# Autodesk Inventor assembly: SE Base Matriz Centelladora DC
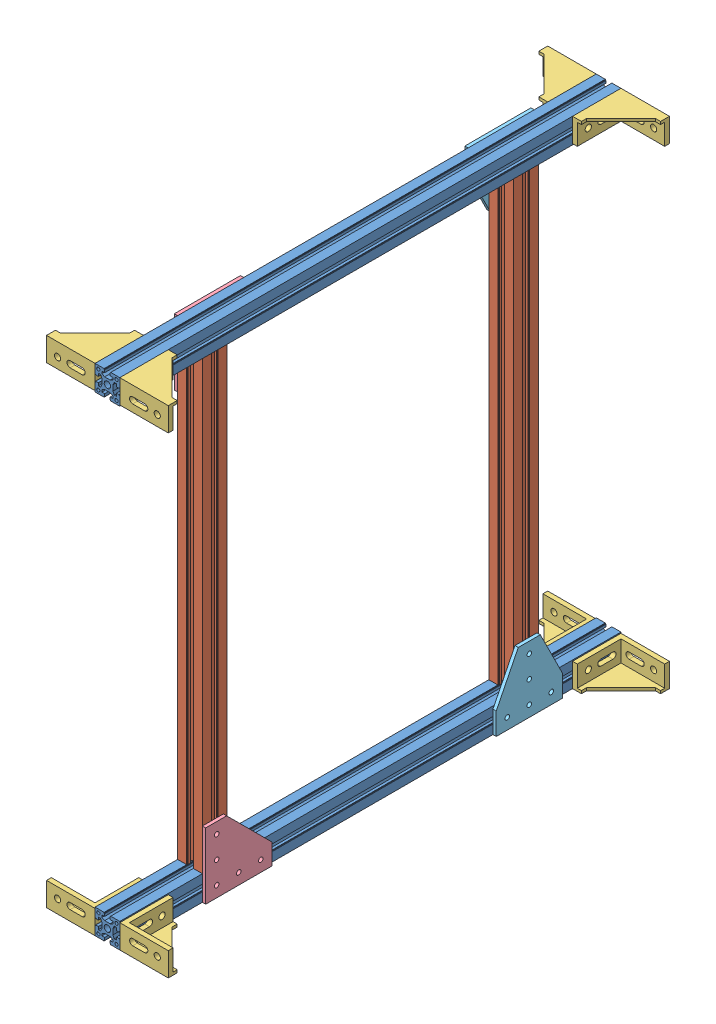
[picture p0: shaded view drawn from the part files that the assembly names]
Saved by Autodesk Inventor 2024.2 (Build 282272000, 272)
## iProperties
Created: 2025-11-13
Part Number: SE Base Matriz Centelladora DC
Document SubType Name: Assembly
Designer: ja.restrepo1
Author: ja.restrepo1
## Documents named in this file (7)
- I:\MICROMECANICA\ALTAS ENERGIAS\Deteccion de Muones\Detectores centelladores\Partes Detector Centellador\SE Base Matriz Centelladora DC\SE Base Matriz Centelladora DC.iam
- I:\MICROMECANICA\ALTAS ENERGIAS\Deteccion de Muones\Detectores centelladores\Partes Detector Centellador\SE Chasis DC\Partes Chasis DC\Perfil 45X45\Perfil 45X45x910.ipt
- I:\MICROMECANICA\ALTAS ENERGIAS\Deteccion de Muones\Detectores centelladores\Partes Detector Centellador\SE Chasis DC\Partes Chasis DC\Perfil 45X45.ipt
- I:\MICROMECANICA\ALTAS ENERGIAS\Deteccion de Muones\Detectores centelladores\Partes Detector Centellador\SE Chasis DC\Partes Chasis DC\Perfil 45X45\Perfil 45X45X810.ipt
- I:\MICROMECANICA\ALTAS ENERGIAS\Deteccion de Muones\Detectores centelladores\Partes Detector Centellador\SE Chasis DC\Partes Chasis DC\Accesorios perfileria\escuadra grande.ipt
- I:\MICROMECANICA\ALTAS ENERGIAS\Deteccion de Muones\Detectores centelladores\Partes Detector Centellador\SE Chasis DC\Partes Chasis DC\Accesorios perfileria\escuadra plana.ipt
- I:\MICROMECANICA\ALTAS ENERGIAS\Deteccion de Muones\Detectores centelladores\Partes Detector Centellador\SE Chasis DC\Partes Chasis DC\Accesorios perfileria\T.ipt
## Components (16 placed, 5 different names)
1. Perfil 45X45x910:1 — Flush:19, Flush:20, Flush:21, Flush:22, Flush:23, Flush:24, Flush:25, Flush:26
2. Perfil 45X45x910:2 — Flush:19, Flush:27, Flush:28, Flush:29, Flush:30
3. Perfil 45X45X810:3
4. Perfil 45X45X810:4 — Flush:20
5. escuadra grande:1 — Flush:23
6. escuadra grande:2 — Flush:24
7. escuadra grande:3 — Flush:30
8. escuadra grande:4 — Flush:26
9. escuadra grande:5 — Flush:28
10. escuadra grande:6 — Flush:27
11. escuadra grande:7 — Flush:25
12. escuadra grande:8 — Flush:29
13. escuadra plana:1
14. T:1
15. T:2
16. escuadra plana:2
## Relationships (47: Flush 30, Mate 17)
- [Flush]: Perfil 45X45X810:3 ↔ Perfil 45X45X810:4
- [Flush]: Perfil 45X45X810:3 ↔ Perfil 45X45X810:4
- [Flush]: Perfil 45X45x910:1 ↔ Perfil 45X45X810:4
- [Mate]: Perfil 45X45x910:2 ↔ Perfil 45X45X810:4
- [Flush]: Perfil 45X45x910:2 ↔ Perfil 45X45X810:4
- [Mate]: Perfil 45X45x910:1 ↔ Perfil 45X45X810:3
- [Mate] (-610 mm): Perfil 45X45X810:3 ↔ Perfil 45X45X810:4
- [Flush]: Perfil 45X45x910:1 ↔ escuadra grande:7
- [Mate]: Perfil 45X45x910:1 ↔ escuadra grande:7
- [Mate]: Perfil 45X45x910:1 ↔ escuadra grande:2
- [Mate]: Perfil 45X45x910:1 ↔ escuadra grande:2
- [Flush]: Perfil 45X45x910:1 ↔ escuadra grande:1
- [Mate]: Perfil 45X45x910:1 ↔ escuadra grande:1
- [Flush]: Perfil 45X45x910:1 ↔ escuadra grande:4
- [Mate]: Perfil 45X45x910:1 ↔ escuadra grande:4
- [Flush]: Perfil 45X45x910:2 ↔ escuadra grande:5
- [Mate]: Perfil 45X45x910:2 ↔ escuadra grande:5
- [Flush]: Perfil 45X45x910:2 ↔ escuadra grande:6
- [Mate]: Perfil 45X45x910:2 ↔ escuadra grande:6
- [Flush]: Perfil 45X45x910:2 ↔ escuadra grande:8
- [Mate]: Perfil 45X45x910:2 ↔ escuadra grande:8
- [Flush]: Perfil 45X45x910:2 ↔ escuadra grande:3
- [Mate]: Perfil 45X45x910:2 ↔ escuadra grande:3
- [Mate]: Perfil 45X45X810:4 ↔ escuadra plana:1
- [Flush]: Perfil 45X45x910:1 ↔ escuadra plana:1
- [Flush]: Perfil 45X45X810:4 ↔ escuadra plana:1
- [Mate]: Perfil 45X45X810:3 ↔ T:2
- [Flush]: Perfil 45X45x910:1 ↔ T:2
- [Mate] (-2.5 mm): Perfil 45X45X810:3 ↔ T:2
- [Mate]: Perfil 45X45X810:3 ↔ T:1
- [Flush]: Perfil 45X45x910:2 ↔ T:1
- [Flush]: T:1 ↔ T:2
- [Mate]: Perfil 45X45X810:4 ↔ escuadra plana:2
- [Flush]: Perfil 45X45x910:2 ↔ escuadra plana:2
- [Flush]: Perfil 45X45X810:4 ↔ escuadra plana:2
- Flush:19: Perfil 45X45x910:1 ↔ Perfil 45X45x910:2
- Flush:20 (150 mm): Perfil 45X45x910:1 ↔ Perfil 45X45X810:4
- Flush:21 (455 mm): Perfil 45X45x910:1
- Flush:22 (455 mm): Perfil 45X45x910:1
- Flush:23: Perfil 45X45x910:1 ↔ escuadra grande:1
- Flush:24: Perfil 45X45x910:1 ↔ escuadra grande:2
- Flush:25: Perfil 45X45x910:1 ↔ escuadra grande:7
- Flush:26: Perfil 45X45x910:1 ↔ escuadra grande:4
- Flush:27: Perfil 45X45x910:2 ↔ escuadra grande:6
- Flush:28: Perfil 45X45x910:2 ↔ escuadra grande:5
- Flush:29: Perfil 45X45x910:2 ↔ escuadra grande:8
- Flush:30: Perfil 45X45x910:2 ↔ escuadra grande:3
